# Autodesk Inventor assembly: climber
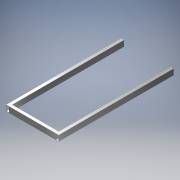
[picture p0: Inventor's stored thumbnail of the model, 180x180]
Saved by Autodesk Inventor 2019.4 (Build 234330000, 330)
## iProperties
Created: 2020-01-07
Part Number: climber
Document SubType Name: Assembly
Designer: Mark
Author: Mark
## Documents named in this file (3)
- C:\Users\Mark\Desktop\7738 Helion Engineering\7738-2020\Elevator Mechanism\climber.iam
- C:\Users\Mark\Desktop\7738 Helion Engineering\7738-2020\Elevator Mechanism\Extrusion Up.ipt
- C:\Users\Mark\Desktop\Extrusion Mid.ipt
## Components (3 placed, 2 different names)
1. Extrusion Up:1 — Mate:1, Flush:1, Flush:2
2. Extrusion Mid:1 — Mate:1, Flush:1, Flush:2, Mate:2, Flush:3, Flush:4
3. Extrusion Up:2 — Mate:2, Flush:3, Flush:4
## Relationships (6: Flush 4, Mate 2)
- Mate:1: Extrusion Up:1 ↔ Extrusion Mid:1
- Flush:1: Extrusion Up:1 ↔ Extrusion Mid:1
- Flush:2: Extrusion Up:1 ↔ Extrusion Mid:1
- Mate:2: Extrusion Mid:1 ↔ Extrusion Up:2
- Flush:3: Extrusion Mid:1 ↔ Extrusion Up:2
- Flush:4: Extrusion Mid:1 ↔ Extrusion Up:2
